# Autodesk Inventor assembly: Assm
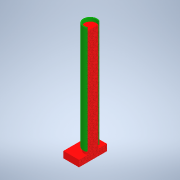
[picture p0: Inventor's stored thumbnail of the model, 180x180]
Saved by Autodesk Inventor 2022 (Build 260153000, 153)
## iProperties
Created: 2022-01-27
Part Number: Assm
Document SubType Name: Assembly
Designer: Administrator
Title: Lab3_Ex0_temp v1
Author: Administrator
## Documents named in this file (3)
- C:\Users\br4ch\M-and-Ms\HW2\Task0\Inventor\Assm.iam
- C:\Users\br4ch\M-and-Ms\HW2\Task0\Inventor\Shtock.ipt
- C:\Users\br4ch\M-and-Ms\HW2\Task0\Inventor\stakan.ipt
## Components (2 placed, 2 different names)
1. Shtock:1 — Cylindrical:1, Mate:1
2. stakan:1 — Cylindrical:1, Mate:1
## Relationships (2: CylindricalJoint 1, Mate 1)
- Cylindrical:1: Shtock:1 ↔ stakan:1
- Mate:1 (6 mm): Shtock:1 ↔ stakan:1
